# Autodesk Inventor assembly: wing
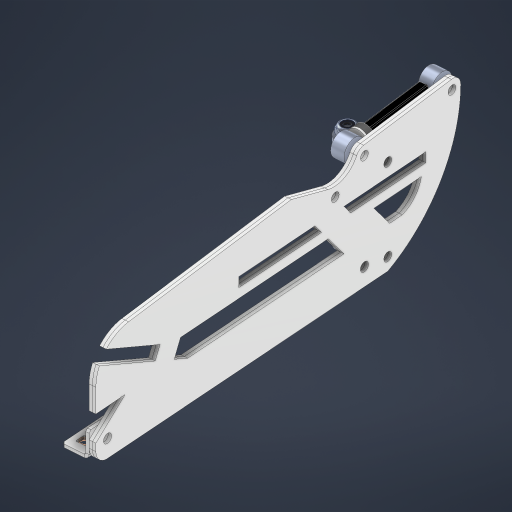
[picture p0: Inventor's stored thumbnail of the model, 512x512]
Saved by Autodesk Inventor 2024 (Build 280153000, 153)
## iProperties
Created: 2023-11-03
Part Number: wing
Document SubType Name: Assembly
Designer: avere
Author: avere
## Documents named in this file (11)
- C:\Users\avere\Documents\rbp_cad\zoomba_v0.1\chassis\wing\wing.iam
- C:\Users\avere\Documents\rbp_cad\zoomba_v0.1\chassis\custom_parts\sled.ipt
- C:\Users\avere\Documents\rbp_cad\VEX-CAD-Inventor-1.41\Motion\Shaft LS\Shaft Collar ipts\Shaft Collar No Screw.ipt
- C:\Users\avere\Documents\rbp_cad\VEX-CAD-Inventor-1.41\Motion\Spacers\Spacer Nylon .375 OD\NSpacer .375 OD x .125.ipt
- C:\Users\avere\Documents\rbp_cad\VEX-CAD-Inventor-1.41\Motion\Spacers\Spacer Nylon .375 OD.ipt
- C:\Users\avere\Documents\rbp_cad\VEX-CAD-Inventor-1.41\Structure\Hardware\Nut Thin Nylock.ipt
- C:\Users\avere\Documents\rbp_cad\VEX-CAD-Inventor-1.41\Structure\Angle\Aluminum 1x1\Alu Angle 1x1x12.ipt
- C:\Users\avere\Documents\rbp_cad\VEX-CAD-Inventor-1.41\Structure\Standoff\Standoff 1.25.ipt
- C:\Users\avere\Documents\rbp_cad\VEX-CAD-Inventor-1.41\Motion\Spacers\Washer Teflon\TWasher .375 OD x .04000.ipt
- C:\Users\avere\Documents\rbp_cad\VEX-CAD-Inventor-1.41\Motion\Spacers\Washer Teflon.ipt
- C:\Users\avere\Documents\rbp_cad\VEX-CAD-Inventor-1.41\Motion\Spacers\Spacer Nylon .375 OD\NSpacer .375 OD x .375.ipt
## Components (13 placed, 8 different names)
1. sled:1 — Insert:10, Mate:4, Insert:11, Insert:15, Mate:5, Insert:16, Insert:17, Insert:18, Mate:7
2. Shaft Collar No Screw:1 — Insert:9, Insert:11
3. Shaft Collar No Screw:2 — Insert:9, Mate:6
4. Shaft Collar No Screw:3 — Mate:5
5. Shaft Collar No Screw:4 — Insert:14, Insert:15
6. Nut Thin Nylock:1
7. Alu Angle 1x1x12:1 — Insert:10, Mate:4
8. NSpacer .375 OD x .125:2 — Insert:12, Insert:13
9. Standoff 1.25:1 — Insert:13
10. TWasher .375 OD x .04000:1 — Insert:12, Insert:14
11. NSpacer .375 OD x .375:3 — Insert:16, Mate:6
12. NSpacer .375 OD x .375:4 — Insert:17
13. sled:2 — Insert:18, Mate:7
## Relationships (16: Insert 11, Mate 5)
- [Mate]: Shaft Collar No Screw:3 ↔ Shaft Collar No Screw:4
- [Insert]: Shaft Collar No Screw:2 ↔ Nut Thin Nylock:1
- Insert:9 (34.925 mm): Shaft Collar No Screw:1 ↔ Shaft Collar No Screw:2
- Insert:10: sled:1 ↔ Alu Angle 1x1x12:1
- Mate:4: sled:1 ↔ Alu Angle 1x1x12:1
- Insert:11 (10.3188 mm): sled:1 ↔ Shaft Collar No Screw:1
- Insert:12: NSpacer .375 OD x .125:2 ↔ TWasher .375 OD x .04000:1
- Insert:13: NSpacer .375 OD x .125:2 ↔ Standoff 1.25:1
- Insert:14: Shaft Collar No Screw:4 ↔ TWasher .375 OD x .04000:1
- Insert:15 (1.5875 mm): sled:1 ↔ Shaft Collar No Screw:4
- Mate:5: sled:1 ↔ Shaft Collar No Screw:3
- Insert:16: sled:1 ↔ NSpacer .375 OD x .375:3
- Insert:17: sled:1 ↔ NSpacer .375 OD x .375:4
- Mate:6: Shaft Collar No Screw:2 ↔ NSpacer .375 OD x .375:3
- Insert:18: sled:1 ↔ sled:2
- Mate:7: sled:1 ↔ sled:2
